# Autodesk Inventor assembly: lowerAssembly
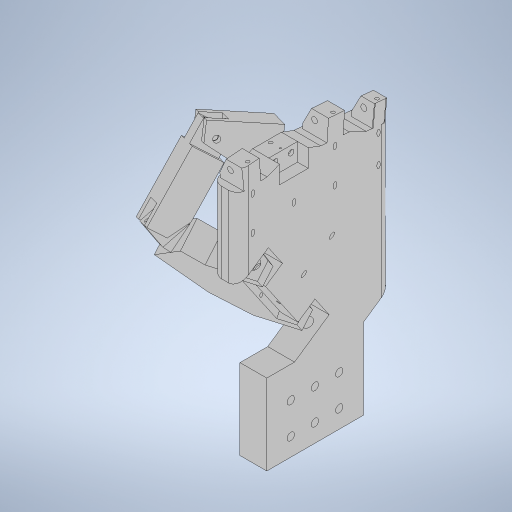
[picture p0: Inventor's stored thumbnail of the model, 512x512]
Saved by Autodesk Inventor 2024 (Build 280153000, 153)
## iProperties
Created: 2024-06-16
Part Number: lowerAssembly
Document SubType Name: Assembly
Designer: omiye
Author: omiye
## Documents named in this file (6)
- C:\Projects\roboticHand\fingerModels\fingerThumb\lowerAssembly.iam
- C:\Projects\roboticHand\fingerModels\normMale.ipt
- C:\Projects\roboticHand\fingerModels\fingerThumb\lower.ipt
- C:\Projects\roboticHand\fingerModels\fingerThumb\middleThumb.ipt
- C:\Projects\roboticHand\fingerModels\fingerThumb\topThumb.ipt
- C:\Projects\roboticHand\fingerModels\palm\palmWithConnectors.ipt
## Components (5 placed, 5 different names)
1. lower:2 — Mate:12, Mate:13, Mate:14, Mate:19, Mate:20
2. normMale:1 — Mate:12, Mate:13, Mate:14, Mate:15, Mate:16
3. middleThumb:1 — Mate:15, Mate:16, Mate:17, Mate:18
4. topThumb:1 — Mate:17, Mate:18
5. palmWithConnectors:1 — Mate:19, Mate:20
## Relationships (9: Mate 9)
- Mate:12: lower:2 ↔ normMale:1
- Mate:13: lower:2 ↔ normMale:1
- Mate:14: lower:2 ↔ normMale:1
- Mate:15: normMale:1 ↔ middleThumb:1
- Mate:16 (0.5 mm): normMale:1 ↔ middleThumb:1
- Mate:17: middleThumb:1 ↔ topThumb:1
- Mate:18 (0.5 mm): middleThumb:1 ↔ topThumb:1
- Mate:19: lower:2 ↔ palmWithConnectors:1
- Mate:20 (1 mm): lower:2 ↔ palmWithConnectors:1
